# Autodesk Inventor assembly: car
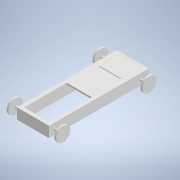
[picture p0: Inventor's stored thumbnail of the model, 180x180]
Saved by Autodesk Inventor 2021 (Build 250183000, 183)
## iProperties
Created: 2021-02-20
Part Number: car
Document SubType Name: Assembly
Designer: bagal
Author: bagal
## Documents named in this file (7)
- C:\Users\bagal\Desktop\inventor models\mousetrap car\car.iam
- C:\Users\bagal\Desktop\inventor models\mousetrap car\mousetrap.ipt
- C:\Users\bagal\Desktop\inventor models\mousetrap car\body_1.ipt
- C:\Users\bagal\Desktop\inventor models\mousetrap car\body_2.ipt
- C:\Users\bagal\Desktop\inventor models\mousetrap car\axle holder.ipt
- C:\Users\bagal\Desktop\inventor models\mousetrap car\axle.ipt
- C:\Users\bagal\Desktop\inventor models\mousetrap car\wheel.ipt
## Components (14 placed, 6 different names)
1. mousetrap:1 — Mate:1, Flush:1, Flush:2, Flush:3, Flush:4, Mate:2
2. body_1:1 — Mate:1, Flush:1, Flush:2, Flush:6, Mate:10, Mate:11, Mate:12, Mate:13
3. body_1:2 — Flush:3, Flush:4, Mate:2, Flush:5, Mate:4, Mate:5, Mate:6, Mate:7, Mate:8, Mate:9
4. body_2:1 — Flush:5, Mate:4, Mate:5, Flush:6
5. axle holder:1 — Mate:8, Mate:9, Mate:21, Mate:22
6. axle holder:2 — Mate:10, Mate:11, Mate:19
7. axle holder:3 — Mate:6, Mate:7, Mate:16, Mate:17
8. axle holder:4 — Mate:12, Mate:13
9. axle:2 — Mate:15, Flush:7, Mate:16, Mate:18
10. wheel:1 — Mate:18, Mate:19
11. wheel:2 — Mate:15, Flush:7, Mate:17
12. axle:3 — Mate:20, Flush:8, Mate:21, Mate:23
13. wheel:3 — Mate:20, Flush:8, Mate:22
14. wheel:4 — Mate:23
## Relationships (29: Mate 21, Flush 8)
- Mate:1: mousetrap:1 ↔ body_1:1
- Flush:1: mousetrap:1 ↔ body_1:1
- Flush:2: mousetrap:1 ↔ body_1:1
- Flush:3: mousetrap:1 ↔ body_1:2
- Flush:4: mousetrap:1 ↔ body_1:2
- Mate:2: mousetrap:1 ↔ body_1:2
- Flush:5: body_1:2 ↔ body_2:1
- Mate:4: body_1:2 ↔ body_2:1
- Mate:5: body_1:2 ↔ body_2:1
- Flush:6: body_1:1 ↔ body_2:1
- Mate:6: body_1:2 ↔ axle holder:3
- Mate:7: body_1:2 ↔ axle holder:3
- Mate:8: body_1:2 ↔ axle holder:1
- Mate:9: body_1:2 ↔ axle holder:1
- Mate:10: body_1:1 ↔ axle holder:2
- Mate:11: body_1:1 ↔ axle holder:2
- Mate:12: body_1:1 ↔ axle holder:4
- Mate:13: body_1:1 ↔ axle holder:4
- Mate:15: axle:2 ↔ wheel:2
- Flush:7: axle:2 ↔ wheel:2
- Mate:16: axle holder:3 ↔ axle:2
- Mate:17: axle holder:3 ↔ wheel:2
- Mate:18: axle:2 ↔ wheel:1
- Mate:19: axle holder:2 ↔ wheel:1
- Mate:20: axle:3 ↔ wheel:3
- Flush:8: axle:3 ↔ wheel:3
- Mate:21: axle holder:1 ↔ axle:3
- Mate:22: axle holder:1 ↔ wheel:3
- Mate:23: axle:3 ↔ wheel:4
